# Autodesk Inventor assembly: workbench
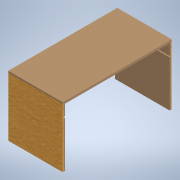
[picture p0: Inventor's stored thumbnail of the model, 180x180]
Saved by Autodesk Inventor 2022 (Build 260153000, 153)
## iProperties
Created: 2022-02-21
Part Number: workbench
Document SubType Name: Assembly
Designer: MarkP
Author: MarkP
## Documents named in this file (6)
- C:\Users\MarkP\Documents\Mark\final\workbench.iam
- C:\Users\MarkP\Documents\Mark\final\desk.ipt
- C:\Users\MarkP\Documents\Mark\final\wallL1.ipt
- C:\Users\MarkP\Documents\Mark\final\wallL2.ipt
- C:\Users\MarkP\Documents\Mark\final\wallL1_MIR.ipt
- C:\Users\MarkP\Documents\Mark\final\wallL2_MIR.ipt
## Components (5 placed, 5 different names)
1. desk:1 — Mate:2, Flush:3, Mate:3
2. wallL1:1 — Flush:1, Mate:1, Flush:2, Flush:3
3. wallL2:1 — Flush:1, Mate:1, Flush:2, Mate:2, Mate:3
4. wallL1_MIR:1 — Flush:4, Mate:4, Flush:5
5. wallL2_MIR:1 — Flush:4, Mate:4, Flush:5
## Relationships (9: Flush 5, Mate 4)
- Flush:1: wallL1:1 ↔ wallL2:1
- Mate:1: wallL1:1 ↔ wallL2:1
- Flush:2: wallL1:1 ↔ wallL2:1
- Mate:2: desk:1 ↔ wallL2:1
- Flush:3: desk:1 ↔ wallL1:1
- Mate:3: desk:1 ↔ wallL2:1
- Flush:4: wallL1_MIR:1 ↔ wallL2_MIR:1
- Mate:4: wallL1_MIR:1 ↔ wallL2_MIR:1
- Flush:5: wallL1_MIR:1 ↔ wallL2_MIR:1
